# Autodesk Inventor assembly: Chessboard Design
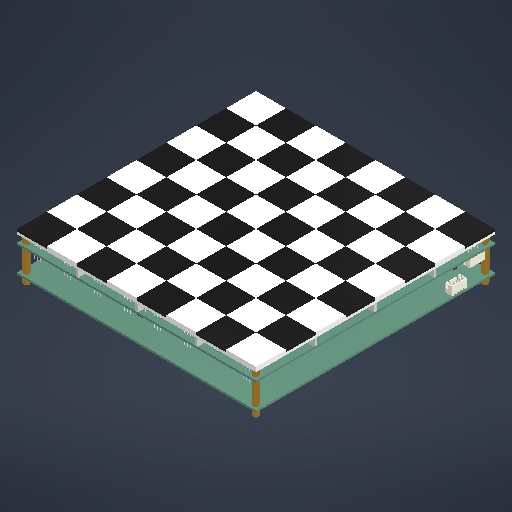
[picture p0: Inventor's stored thumbnail of the model, 512x512]
Saved by Autodesk Inventor 2026 (Build 300175000, 175)
## iProperties
Created: 2025-04-19
Part Number: Chessboard Design
Document SubType Name: Assembly
Designer: ckyiu
Author: ckyiu
## Documents named in this file (4)
- C:\Users\ckyiu\Documents\Projects\Chessboard-Design\Chessboard Design.iam
- C:\Users\ckyiu\Documents\Projects\Chessboard-Design\Assemblies\Chessboard Bottom.iam
- C:\Users\ckyiu\Documents\Projects\Chessboard-Design\Parts\Square Holder Support.ipt
- C:\Users\ckyiu\Documents\Projects\Chessboard-Design\Assemblies\Chessboard Top.iam
## Components (3 placed, 3 different names)
1. Chessboard Bottom:1 [sub-assembly] — Mate:1, Flush:1, Flush:2, Flush:3, Flush:4
2. Square Holder Support:1 — Mate:1, Flush:1, Flush:2, Mate:2
3. Chessboard Top:1 [sub-assembly] — Mate:2, Flush:3, Flush:4
## Relationships (6: Flush 4, Mate 2)
- Mate:1: Chessboard Bottom:1 ↔ Square Holder Support:1
- Flush:1: Chessboard Bottom:1 ↔ Square Holder Support:1
- Flush:2: Chessboard Bottom:1 ↔ Square Holder Support:1
- Mate:2: Square Holder Support:1 ↔ Chessboard Top:1
- Flush:3: Chessboard Bottom:1 ↔ Chessboard Top:1
- Flush:4: Chessboard Bottom:1 ↔ Chessboard Top:1
